# Autodesk Inventor assembly: motor_spool
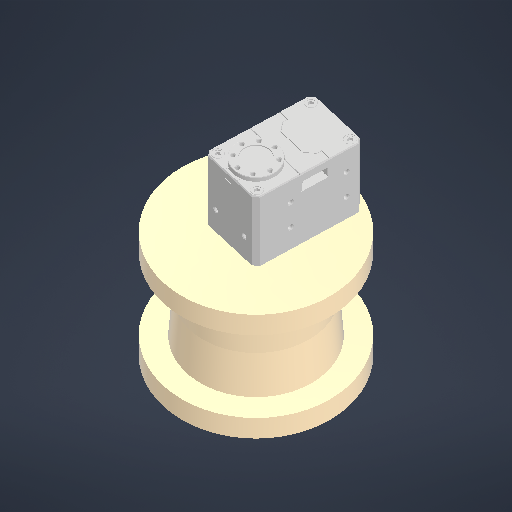
[picture p0: Inventor's stored thumbnail of the model, 512x512]
Saved by Autodesk Inventor 2026.2 (Build 302298010, 298A)
## iProperties
Created: 2026-03-01
Part Number: motor_spool
Document SubType Name: Assembly
Designer: Luke
Author: Luke
## Documents named in this file (3)
- C:\Users\Luke\OneDrive - Heriot-Watt University\Desktop\Robot Mech Sys\GroupProject\CAD\sub_assemblies\motor_spool_sub_assem.iam
- C:\Users\Luke\OneDrive - Heriot-Watt University\Desktop\Robot Mech Sys\GroupProject\CAD\parts\spool.ipt
- C:\Users\Luke\OneDrive - Heriot-Watt University\Desktop\Robot Mech Sys\GroupProject\CAD\parts\motor_imported_Simplify_1.ipt
## Components (2 placed, 2 different names)
1. spool:1 — Mate:1, Mate:2
2. motor_imported_Simplify_1:1 — Mate:1, Mate:2
## Relationships (2: Mate 2)
- Mate:1: spool:1 ↔ motor_imported_Simplify_1:1
- Mate:2: spool:1 ↔ motor_imported_Simplify_1:1
